# Autodesk Inventor assembly: frame
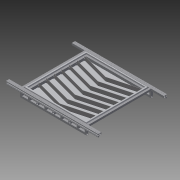
[picture p0: Inventor's stored thumbnail of the model, 180x180]
Saved by Autodesk Inventor 2013 (Build 170138000, 138)
## iProperties
Created: 2012-10-19
Part Number: frame
Document SubType Name: Assembly
Designer: Istvan
Mass: 30866 g
Surface Area: 132817 cm^2
Volume: 17609.3 cm^3
Density: 1.75282 g/cm^3
Author: Istvan
## Documents named in this file (9)
- E:\GitHub\Crown-Fire\CAD\Frame\frame.iam
- E:\GitHub\Crown-Fire\CAD\Frame\Table\table.iam
- E:\GitHub\Crown-Fire\CAD\Frame\Supports\supports.iam
- E:\GitHub\Crown-Fire\CAD\GantryMount\rack.ipt
- E:\GitHub\Crown-Fire\CAD\GantryMount\cChannel.ipt
- D:\GitHub\Crown-Fire\CAD\Templates\cChannel2x1.ipt
- E:\GitHub\Crown-Fire\CAD\Templates\vee-track.ipt
- E:\GitHub\Crown-Fire\CAD\GantryMount\y-vee-track.ipt
- E:\GitHub\Crown-Fire\CAD\GantryMount\veeTrackMount.ipt
## Components (10 placed, 6 different names)
1. table:1 [sub-assembly] — Mate:5, Mate:18, Mate:19
2. supports:1 [sub-assembly] — Mate:5, Mate:7, Mate:8, Flush:1, Flush:2, Flush:3, Flush:4, Mate:18, Mate:19
3. rack:1 — Flush:5, Mate:15, Flush:9
4. rack:2 — Flush:6, Mate:14, Flush:10
5. cChannel:1 — Mate:8, Flush:2, Flush:4, Flush:5, Mate:15, Flush:9, Mate:22, Mate:23, Flush:11
6. cChannel:2 — Mate:7, Flush:1, Flush:3, Flush:6, Mate:14, Flush:10, Mate:26, Flush:14, Mate:29
7. y-vee-track:1 — Flush:15, Mate:27, Mate:28
8. y-vee-track:2 — Mate:24, Flush:13, Mate:25
9. veeTrackMount:1 — Mate:22, Mate:23, Flush:11, Mate:24, Flush:13, Mate:25
10. veeTrackMount:2 — Mate:26, Flush:14, Flush:15, Mate:27, Mate:28, Mate:29
## Relationships (27: Mate 15, Flush 12)
- Mate:5: table:1 ↔ supports:1
- Mate:7: supports:1 ↔ cChannel:2
- Mate:8: supports:1 ↔ cChannel:1
- Flush:1: supports:1 ↔ cChannel:2
- Flush:2: supports:1 ↔ cChannel:1
- Flush:3: supports:1 ↔ cChannel:2
- Flush:4: supports:1 ↔ cChannel:1
- Flush:5: rack:1 ↔ cChannel:1
- Flush:6: rack:2 ↔ cChannel:2
- Mate:14: rack:2 ↔ cChannel:2
- Mate:15: rack:1 ↔ cChannel:1
- Mate:18 (12.7 mm): table:1 ↔ supports:1
- Mate:19 (12.7 mm): table:1 ↔ supports:1
- Flush:9 (6.35 mm): rack:1 ↔ cChannel:1
- Flush:10 (6.35 mm): rack:2 ↔ cChannel:2
- Mate:22: cChannel:1 ↔ veeTrackMount:1
- Mate:23: cChannel:1 ↔ veeTrackMount:1
- Flush:11: cChannel:1 ↔ veeTrackMount:1
- Mate:24: y-vee-track:2 ↔ veeTrackMount:1
- Flush:13: y-vee-track:2 ↔ veeTrackMount:1
- Mate:25: y-vee-track:2 ↔ veeTrackMount:1
- Mate:26: cChannel:2 ↔ veeTrackMount:2
- Flush:14: cChannel:2 ↔ veeTrackMount:2
- Flush:15: y-vee-track:1 ↔ veeTrackMount:2
- Mate:27: y-vee-track:1 ↔ veeTrackMount:2
- Mate:28: y-vee-track:1 ↔ veeTrackMount:2
- Mate:29: cChannel:2 ↔ veeTrackMount:2
